# Autodesk Inventor assembly: RT_ELE_003_350mmGutter
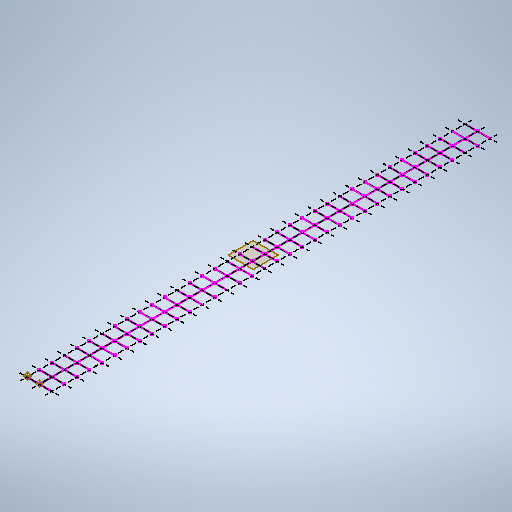
[picture p0: Inventor's stored thumbnail of the model, 512x512]
Saved by Autodesk Inventor 2025.3 (Build 293356000, 356)
## iProperties
Created: 2026-07-30
Part Number: RT_ELE_003_350mmGutter
Document SubType Name: Assembly
Designer: louis
Author: louis
## Documents named in this file (3)
- C:\Users\louis\OneDrive\Desktop\R_Trident\02_CAD\04_Subassemblies\RT_ELE_003_350mmGutter.iam
- C:\Users\louis\OneDrive\Desktop\R_Trident\02_CAD\01_Standard_Parts\04_ELE_Electrical_Automation\Cable channel 60x25\Cable channel 60x25x350.ipt
- C:\Users\louis\OneDrive\Desktop\R_Trident\02_CAD\04_Subassemblies\RT_ELE_003_350mmGutter\AIP\Cable and Harness\RT_ELE_003_350mmGutter.Harness1.iam
## Components (2 placed, 2 different names)
1. Cable channel 60x25x350:1 — Flush:1
2. Harness1 [sub-assembly]
## Relationships (1: Flush 1)
- Flush:1: Cable channel 60x25x350:1
